# Autodesk Inventor assembly: TS_V1_Fallmagazin_gesamt
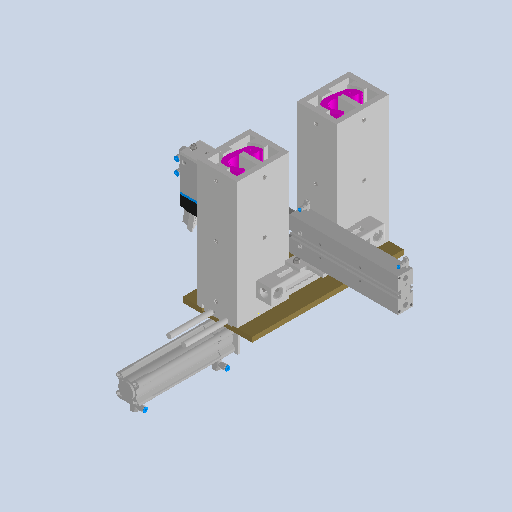
[picture p0: Inventor's stored thumbnail of the model, 512x512]
Saved by Autodesk Inventor 2025.2 (Build 292293000, 293)
## iProperties
Created: 2025-06-10
Part Number: TS_V1_Fallmagazin_gesamt
Document SubType Name: Assembly
Designer: tino
Author: tino
## Documents named in this file (36)
- D:\Useless_Box\CAD-Paspa\Useless Box\Eigene Bauteile\Fallmagazin\TS_V1_Fallmagazin_gesamt.iam
- D:\Useless_Box\CAD-Paspa\Useless Box\Eigene Bauteile\Fallmagazin\TS_V1_Fallmagazin_Boden_int.ipt
- D:\Useless_Box\CAD-Paspa\Useless Box\Eigene Bauteile\Fallmagazin\TS_V1_Fallmagazin_Wandung_int.ipt
- D:\Useless_Box\CAD-Paspa\Useless Box\Eigene Bauteile\Fallmagazin\TS_V1_Fallmagazin_Leitbleche_vorne_int.ipt
- D:\Useless_Box\CAD-Paspa\Useless Box\_Useless_Box\Finger.ipt
- D:\Useless_Box\CAD-Paspa\Useless Box\Eigene Bauteile\Fallmagazin\TS_V1_Fallmagazin_Schieber.iam
- D:\Useless_Box\CAD-Paspa\Useless Box\Kaufteile\Festo_Normzylinder_100\1376426 DSBC-32-100-PPVA-N3---(0).iam
- D:\Useless_Box\CAD-Paspa\Useless Box\Standart Bauteile\ISO 4762 - M4 x 12ISO.ipt
- D:\Useless_Box\CAD-Paspa\Useless Box\Standart Bauteile\ISO 4762 - M4 x 16ISO.ipt
- D:\Useless_Box\CAD-Paspa\Useless Box\Eigene Bauteile\Fallmagazin\TS_V1_Fallmagazin_Zylinderanbindung_int.ipt
- D:\Useless_Box\CAD-Paspa\Useless Box\Eigene Bauteile\Fallmagazin\TS_V1_Fallmagazin_Stopper_int.ipt
- D:\Useless_Box\CAD-Paspa\Useless Box\Eigene Bauteile\Fallmagazin\TS_V1_Fallmagazin_Zylinderhalter_int.ipt
- D:\Useless_Box\CAD-Paspa\Useless Box\Standart Bauteile\ISO 4762 - M5 x 8ISO.ipt
- D:\Useless_Box\CAD-Paspa\Useless Box\Standart Bauteile\ISO 4762 - M5 x 20ISO.ipt
- D:\Useless_Box\CAD-Paspa\Useless Box\Standart Bauteile\DIN EN ISO 2338 - 4 m6 x 10.ipt
- D:\Useless_Box\CAD-Paspa\Useless Box\Standart Bauteile\DIN 7991 - M5x12.ipt
- D:\Useless_Box\CAD-Paspa\Useless Box\Eigene Bauteile\Fallmagazin\TS_V1_Fallmagazin_Schieberanbindung_int.ipt
- D:\Useless_Box\CAD-Paspa\Useless Box\Eigene Bauteile\Fallmagazin\TS_V1_Fallmagazin_Verbindungsstange_int.ipt
- D:\Useless_Box\CAD-Paspa\Useless Box\Kaufteile\Festo_Fuehrungszylinder150_DFM_16\529120 DFM-16-150-B-P-A-KF---(0).iam
- D:\Useless_Box\CAD-Paspa\Useless Box\Kaufteile\DHRS-32-A - Kopie\AIS2024\1310164 DHRS-32-A---(0).iam
- D:\Useless_Box\CAD-Paspa\Useless Box\Eigene Bauteile\TS_Adapter_Greifer_int.ipt
- D:\Useless_Box\CAD-Paspa\Useless Box\Standart Bauteile\ISO 4762 - M4 x 10ISO.ipt
- D:\Useless_Box\CAD-Paspa\Useless Box\Eigene Bauteile\TS_Halterung_Fuehrungszylinder_int.ipt
- D:\Useless_Box\CAD-Paspa\Useless Box\Kaufteile\Rexroth_Profil+Winkel_30x30\Rexroth_30x30_Wuerfel\Rexroth_30x30_Wuerfel\Rexroth_30x30_Wuerfel.ipt
- D:\Useless_Box\CAD-Paspa\Useless Box\Kaufteile\Rexroth_Profil+Winkel_30x30\Rexroth_30x30_200_ext\Rexroth_30x30_200_ext\Rexroth_30x30_200_ext.ipt
- D:\Useless_Box\CAD-Paspa\Useless Box\Standart Bauteile\DIN 7991 - M8x16.ipt
- D:\Useless_Box\CAD-Paspa\Useless Box\Standart Bauteile\DIN 934 - M5 x 0,8.ipt
- D:\Useless_Box\CAD-Paspa\Useless Box\Standart Bauteile\ISO 4762 - M6 x 12ISO.ipt
- D:\Useless_Box\CAD-Paspa\Useless Box\Kaufteile\Rexroth_Hammermuttern\Rexroth_Hammermutter_8_M6\Rexroth_Hammermutter_8_M6\Rexroth_Hammermutter_8_M6.ipt
- D:\Useless_Box\CAD-Paspa\Useless Box\Standart Bauteile\DIN 913 - M5 x 6.ipt
- D:\Useless_Box\CAD-Paspa\Useless Box\Eigene Bauteile\JH_Greifer_Unterlegscheibe\Kaufteile\Drosselrückschlagventil\175043 GRLZ-M3-QS-3.ipt
- D:\Useless_Box\CAD-Paspa\Useless Box\Eigene Bauteile\JH_Greifer_Unterlegscheibe\Kaufteile\Drosselrückschlagventil\193143 GRLA-1_8-QS-4-D.ipt
- D:\Useless_Box\CAD-Paspa\Useless Box\Standart Bauteile\DIN 6912 - M4 x 10.ipt
- C:\Users\Erik\Documents\Inventor\Content Center Files\R2025\de-DE\DIN ISO 8734(1)\ISO 8734 - 4 x 10 - ADIN EN.ipt
- D:\Useless_Box\CAD-Paspa\Useless Box\Standart Bauteile\DIN EN ISO 4762 - M5 x 10.ipt
- D:\Useless_Box\CAD-Paspa\Useless Box\Standart Bauteile\DIN 125 - A 5,3.ipt
## Components (206 placed, 35 different names)
1. TS_V1_Fallmagazin_Boden_int:1 — Passend:16, Passend:17, Passend:21, Passend:23, Passend:25, Passend:26, Passend:30, Passend:43, Passend:44, Passend:45, Passend:46, Fluchtend:18, Passend:84, Passend:85, Passend:86, Passend:87, Passend:94, Passend:96, Passend:97, Fluchtend:19, Fluchtend:20, Passend:121, Winkel:11, Winkel:12
2. TS_V1_Fallmagazin_Wandung_int:2 — Passend:7, Passend:8, Fluchtend:4, Winkel:1, Winkel:2, Passend:16, Passend:17, Passend:35, Passend:36, Passend:37, Passend:38, Passend:39, Passend:40, Passend:41, Passend:42, Winkel:3, Passend:130
3. TS_V1_Fallmagazin_Leitbleche_vorne_int:1 — Passend:7, Passend:8, Fluchtend:4, Tangential:2, Tangential:5, Fluchtend:12
4. TS_V1_Fallmagazin_Schieber:1 [sub-assembly] — Passend:21, Passend:25, Passend:26, Passend:53, Passend:61, Passend:62, Passend:63, Passend:64, Passend:106, Tangential:6
5. TS_V1_Fallmagazin_Schieber:2 [sub-assembly] — Passend:23, Passend:30, Passend:65, Passend:66, Passend:67, Passend:101, Passend:103, Passend:107
6. 1376426 DSBC-32-100-PPVA-N3---(0):1 [sub-assembly] — Fluchtend:18, Passend:68, Passend:69, Passend:92, Passend:93, Passend:99, Einfügen:1, Passend:159
7. TS_V1_Fallmagazin_Wandung_int:3 — Passend:45, Passend:46, Passend:47, Fluchtend:14, Passend:48, Passend:132, Passend:137, Passend:138
8. TS_V1_Fallmagazin_Leitbleche_vorne_int:2 — Passend:47, Fluchtend:14, Passend:48
9. TS_V1_Fallmagazin_Zylinderanbindung_int:1 — Passend:53, Passend:99, Winkel:4, Passend:104, Passend:108, Passend:110, Passend:144
10. TS_V1_Fallmagazin_Stopper_int:1 — Passend:61, Passend:62, Winkel:3
11. TS_V1_Fallmagazin_Stopper_int:2 — Passend:63, Passend:64
12. TS_V1_Fallmagazin_Stopper_int:3 — Passend:65, Fluchtend:16, Passend:67
13. TS_V1_Fallmagazin_Stopper_int:4 — Passend:66, Fluchtend:16
14. TS_V1_Fallmagazin_Zylinderhalter_int:1 — Passend:68, Passend:69, Passend:71, Passend:72, Passend:90, Passend:91, Passend:93, Passend:95, Passend:97
15. DIN 7991 M5x12:1 — Passend:106, Tangential:6, Passend:108
16. DIN 7991 M5x12:2 — Passend:101, Passend:107, Passend:109
17. TS_V1_Fallmagazin_Schieberanbindung_int:1 — Winkel:4, Passend:103, Passend:105, Passend:109, Passend:142
18. TS_V1_Fallmagazin_Verbindungsstange_int:1 — Passend:104, Passend:105, Winkel:5, Passend:110, Passend:141, Passend:143
19. 529120 DFM-16-150-B-P-A-KF---(0):1 [sub-assembly] — Fluchtend:19, Winkel:6, Fluchtend:21, Passend:116, Passend:117, Passend:120, Passend:121, Passend:122, Passend:123, Passend:124, Winkel:7, Winkel:8, Passend:157, Passend:158, Winkel:10
20. 1310164 DHRS-32-A---(0):1 [sub-assembly] — Fluchtend:20, Fluchtend:21, Passend:113, Passend:118, Passend:119, Passend:153, Passend:155, Passend:156, Einfügen:2, Einfügen:3, Einfügen:4, Einfügen:5, Einfügen:6, Einfügen:7, Passend:162
21. TS_Adapter_Greifer_int:1 — Passend:113, Passend:114, Passend:115, Passend:118, Passend:119, Passend:120, Passend:153, Passend:154, Fluchtend:26, Winkel:9, Passend:163
22. TS_Halterung_Fuehrungszylinder_int:1 — Passend:122, Passend:123, Passend:124, Passend:135, Passend:145, Passend:146, Passend:147, Passend:148, Passend:150, Passend:151, Passend:152
23. Rexroth_30x30_Wuerfel:1 — Passend:130, Passend:134, Fluchtend:24, Fluchtend:25, Passend:136, Tangential:7, Passend:139, Tangential:9
24. Rexroth_30x30_Wuerfel:2 — Passend:132, Passend:133, Fluchtend:22, Fluchtend:23, Passend:137, Tangential:8, Passend:140, Tangential:10
25. Rexroth_30x30_170_ext:1 — Passend:133, Fluchtend:22, Fluchtend:23, Passend:134, Fluchtend:24, Fluchtend:25, Passend:135, Tangential:11, Tangential:12
26. DIN 7991 M8x16:3 — Passend:136, Tangential:7
27. DIN 7991 M8x16:4 — Passend:138, Tangential:8
28. DIN 7991 M8x16:5 — Passend:139, Tangential:9
29. DIN 7991 M8x16:6 — Passend:140, Tangential:10
30. DIN 934 - M5 x 0,8:1 — Passend:141, Passend:142
31. DIN 934 - M5 x 0,8:2 — Passend:143, Passend:144
32. ISO 4762 - M6 x 12ISO:1 — Passend:147, Passend:148, Passend:149
33. Rexroth_Hammermutter_8_M6:1 — Winkel:7, Tangential:11, Passend:149
34. Rexroth_Hammermutter_8_M6:2 — Winkel:8, Tangential:12, Passend:150
35. ISO 4762 - M6 x 12ISO:2 — Passend:151, Passend:152
36. DIN 913 - M5 x 6:1 — Passend:154, Fluchtend:26
37. 193143 GRLA-1_8-QS-4-D:3 — Einfügen:1, Winkel:11
38. 193143 GRLA-1_8-QS-4-D:4 — Passend:159, Winkel:12
39. DIN 6912 - M4 x 10:1 — Einfügen:2
40. DIN 6912 - M4 x 10:2 — Einfügen:3
41. DIN 6912 - M4 x 10:3 — Einfügen:4
42. DIN 6912 - M4 x 10:4 — Einfügen:5
43. DIN EN ISO 8734 4 x 10 - A:1 — Einfügen:7
44. DIN EN ISO 8734 4 x 10 - A:2 — Einfügen:6
45. Finger:1 — Winkel:1, Tangential:2, Tangential:5, Winkel:2, Fluchtend:12
46. Finger:2
47. Finger:3
48. Finger:4
49. Finger:5
50. Finger:6
51. Finger:7
52. Finger:8
53. Finger:9
54. Finger:10
55. Finger:11
56. Finger:12
57. Finger:13
58. Finger:14
59. Finger:15
60. Finger:16
61. Finger:17
62. Finger:18
63. Finger:19
64. Finger:20
65. Finger:21
66. Finger:22
67. Finger:23
68. Finger:24
69. Finger:25
70. Finger:26
71. Finger:27
72. Finger:28
73. Finger:29
74. Finger:30
75. Finger:31
76. Finger:32
77. Finger:33
78. Finger:34
79. Finger:35
80. Finger:36
81. Finger:37
82. Finger:38
83. Finger:39
84. Finger:40
85. Finger:41
86. Finger:42
87. Finger:43
88. Finger:44
89. Finger:45
90. Finger:46
91. Finger:47
92. Finger:48
93. Finger:49
94. Finger:50
95. Finger:51
96. Finger:52
97. Finger:53
98. Finger:54
99. Finger:55
100. Finger:56
101. Finger:57
102. Finger:58
103. Finger:59
104. Finger:60
105. Finger:61
106. Finger:62
107. Finger:63
108. Finger:64
109. Finger:65
110. Finger:66
111. Finger:67
112. Finger:68
113. Finger:69
114. Finger:70
115. Finger:71
116. Finger:72
117. Finger:73
118. Finger:74
119. Finger:75
120. Finger:76
121. Finger:77
122. Finger:78
123. Finger:79
124. Finger:80
125. Finger:81
126. Finger:82
127. Finger:83
128. Finger:84
129. Finger:85
130. Finger:86
131. Finger:87
132. Finger:88
133. Finger:89
134. Finger:90
135. Finger:91
136. Finger:92
137. Finger:93
138. Finger:94
139. Finger:95
140. Finger:96
141. Finger:97
142. Finger:98
143. ISO 4762 M5 x 8:1 — Passend:71, Passend:72, Passend:96
144. ISO 4762 M5 x 8:2
145. ISO 4762 M5 x 8:3 — Passend:94
146. ISO 4762 M5 x 8:4
147. ISO 4762 M5 x 20:1 — Passend:92, Passend:95
148. ISO 4762 M5 x 20:2 — Passend:91
149. ISO 4762 M5 x 20:3 — Passend:90
150. ISO 4762 M5 x 20:4
151. ISO 4762 M4 x 10:1 — Passend:114, Passend:115, Passend:116
152. ISO 4762 M4 x 10:2 — Passend:117
153. ISO 4762 M4 x 10:3
154. ISO 4762 M4 x 10:4
155. DIN EN ISO 2338 4 m6 x 10:1 — Passend:84, Passend:85
156. DIN EN ISO 2338 4 m6 x 10:2 — Passend:86, Passend:87
157. DIN EN ISO 2338 4 m6 x 10:3
158. DIN EN ISO 2338 4 m6 x 10:4
159. ISO 4762 M4 x 10:5 — Passend:145, Passend:146
160. ISO 4762 M4 x 10:6
161. ISO 4762 M4 x 10:7
162. ISO 4762 M4 x 10:8
163. 193143 GRLA-1_8-QS-4-D:1 — Passend:155, Passend:156, Winkel:9
164. 193143 GRLA-1_8-QS-4-D:2
165. 175043 GRLZ-M3-QS-3:1 — Passend:157, Passend:158, Winkel:10
166. 175043 GRLZ-M3-QS-3:2
167. DIN 125 - A 5,3:1 — Passend:163
168. DIN EN ISO 4762 - M5 x 10:1 — Passend:162
169. DIN 125 - A 5,3:2
170. DIN EN ISO 4762 - M5 x 10:2
171. ISO 4762 M4 x 12:1 — Passend:35, Passend:36
172. ISO 4762 M4 x 12:2
173. ISO 4762 M4 x 12:3
174. ISO 4762 M4 x 12:4 — Passend:37, Passend:38
175. ISO 4762 M4 x 12:5
176. ISO 4762 M4 x 12:6
177. ISO 4762 M4 x 12:7 — Passend:39, Passend:40
178. ISO 4762 M4 x 12:8
179. ISO 4762 M4 x 12:9
180. ISO 4762 M4 x 12:10 — Passend:41, Passend:42
181. ISO 4762 M4 x 12:11
182. ISO 4762 M4 x 12:12
183. ISO 4762 M4 x 16:1 — Passend:43, Passend:44
184. ISO 4762 M4 x 16:2
185. ISO 4762 M4 x 16:3
186. ISO 4762 M4 x 16:4
187. ISO 4762 M4 x 16:5
188. ISO 4762 M4 x 16:6
189. ISO 4762 M4 x 12:13
190. ISO 4762 M4 x 12:14
191. ISO 4762 M4 x 12:15
192. ISO 4762 M4 x 12:16
193. ISO 4762 M4 x 12:17
194. ISO 4762 M4 x 12:18
195. ISO 4762 M4 x 12:19
196. ISO 4762 M4 x 12:20
197. ISO 4762 M4 x 12:21
198. ISO 4762 M4 x 12:22
199. ISO 4762 M4 x 12:23
200. ISO 4762 M4 x 12:24
201. ISO 4762 M4 x 16:7
202. ISO 4762 M4 x 16:8
203. ISO 4762 M4 x 16:9
204. ISO 4762 M4 x 16:10
205. ISO 4762 M4 x 16:11
206. ISO 4762 M4 x 16:12
## Component patterns: (2 elements), (98 elements, first: Finger:1), (4 elements, first: ISO 4762 M5 x 8:1), (4 elements, first: ISO 4762 M5 x 20:1), (4 elements, first: ISO 4762 M4 x 10:1), (2 elements, first: DIN EN ISO 2338 4 m6 x 10:1 + DIN EN ISO 2338 4 m6 x 10:2), (4 elements, first: ISO 4762 M4 x 10:5), (2 elements, first: 193143 GRLA-1_8-QS-4-D:1), (2 elements, first: 175043 GRLZ-M3-QS-3:1), (2 elements, first: DIN 125 - A 5,3:1 + DIN EN ISO 4762 - M5 x 10:1), (3 elements, first: ISO 4762 M4 x 12:1), (3 elements, first: ISO 4762 M4 x 12:4), (3 elements, first: ISO 4762 M4 x 12:7), (3 elements, first: ISO 4762 M4 x 12:10), (6 elements, first: ISO 4762 M4 x 16:1), Komponentenanordnung 2:2 (3 elements), Komponentenanordnung 3:2 (3 elements), Komponentenanordnung 4:2 (3 elements), Komponentenanordnung 5:2 (3 elements), Komponentenanordnung 6:2 (6 elements)
## Relationships (143: Mate 102, Flush 13, Angle 12, Tangent 9, Insert 7)
- Passend:7 [Mate]: TS_V1_Fallmagazin_Wandung_int:2 ↔ TS_V1_Fallmagazin_Leitbleche_vorne_int:1
- Passend:8 [Mate]: TS_V1_Fallmagazin_Wandung_int:2 ↔ TS_V1_Fallmagazin_Leitbleche_vorne_int:1
- Fluchtend:4 [Flush]: TS_V1_Fallmagazin_Wandung_int:2 ↔ TS_V1_Fallmagazin_Leitbleche_vorne_int:1
- Winkel:1 [Angle] (0 deg): TS_V1_Fallmagazin_Wandung_int:2 ↔ Finger:1
- Tangential:2: TS_V1_Fallmagazin_Leitbleche_vorne_int:1 ↔ Finger:1
- Tangential:5: TS_V1_Fallmagazin_Leitbleche_vorne_int:1 ↔ Finger:1
- Winkel:2 [Angle] (0 deg): TS_V1_Fallmagazin_Wandung_int:2 ↔ Finger:1
- Passend:16 [Mate]: TS_V1_Fallmagazin_Boden_int:1 ↔ TS_V1_Fallmagazin_Wandung_int:2
- Passend:17 [Mate]: TS_V1_Fallmagazin_Boden_int:1 ↔ TS_V1_Fallmagazin_Wandung_int:2
- Passend:21 [Mate]: TS_V1_Fallmagazin_Boden_int:1 ↔ TS_V1_Fallmagazin_Schieber:1
- Passend:23 [Mate]: TS_V1_Fallmagazin_Boden_int:1 ↔ TS_V1_Fallmagazin_Schieber:2
- Passend:25 [Mate]: TS_V1_Fallmagazin_Boden_int:1 ↔ TS_V1_Fallmagazin_Schieber:1
- Passend:26 [Mate]: TS_V1_Fallmagazin_Boden_int:1 ↔ TS_V1_Fallmagazin_Schieber:1
- Passend:30 [Mate]: TS_V1_Fallmagazin_Boden_int:1 ↔ TS_V1_Fallmagazin_Schieber:2
- Passend:35 [Mate]: TS_V1_Fallmagazin_Wandung_int:2 ↔ ISO 4762 M4 x 12:1
- Passend:36 [Mate]: TS_V1_Fallmagazin_Wandung_int:2 ↔ ISO 4762 M4 x 12:1
- Passend:37 [Mate]: TS_V1_Fallmagazin_Wandung_int:2 ↔ ISO 4762 M4 x 12:4
- Passend:38 [Mate]: TS_V1_Fallmagazin_Wandung_int:2 ↔ ISO 4762 M4 x 12:4
- Passend:39 [Mate]: TS_V1_Fallmagazin_Wandung_int:2 ↔ ISO 4762 M4 x 12:7
- Passend:40 [Mate]: TS_V1_Fallmagazin_Wandung_int:2 ↔ ISO 4762 M4 x 12:7
- Passend:41 [Mate]: TS_V1_Fallmagazin_Wandung_int:2 ↔ ISO 4762 M4 x 12:10
- Passend:42 [Mate]: TS_V1_Fallmagazin_Wandung_int:2 ↔ ISO 4762 M4 x 12:10
- Passend:43 [Mate]: TS_V1_Fallmagazin_Boden_int:1 ↔ ISO 4762 M4 x 16:1
- Passend:44 [Mate]: TS_V1_Fallmagazin_Boden_int:1 ↔ ISO 4762 M4 x 16:1
- Fluchtend:12 [Flush]: TS_V1_Fallmagazin_Leitbleche_vorne_int:1 ↔ Finger:1
- Passend:45 [Mate]: TS_V1_Fallmagazin_Boden_int:1 ↔ TS_V1_Fallmagazin_Wandung_int:3
- Passend:46 [Mate]: TS_V1_Fallmagazin_Boden_int:1 ↔ TS_V1_Fallmagazin_Wandung_int:3
- Passend:47 [Mate]: TS_V1_Fallmagazin_Wandung_int:3 ↔ TS_V1_Fallmagazin_Leitbleche_vorne_int:2
- Fluchtend:14 [Flush]: TS_V1_Fallmagazin_Wandung_int:3 ↔ TS_V1_Fallmagazin_Leitbleche_vorne_int:2
- Passend:48 [Mate]: TS_V1_Fallmagazin_Wandung_int:3 ↔ TS_V1_Fallmagazin_Leitbleche_vorne_int:2
- Passend:53 [Mate]: TS_V1_Fallmagazin_Schieber:1 ↔ TS_V1_Fallmagazin_Zylinderanbindung_int:1
- Passend:61 [Mate]: TS_V1_Fallmagazin_Schieber:1 ↔ TS_V1_Fallmagazin_Stopper_int:1
- Passend:62 [Mate]: TS_V1_Fallmagazin_Schieber:1 ↔ TS_V1_Fallmagazin_Stopper_int:1
- Passend:63 [Mate]: TS_V1_Fallmagazin_Schieber:1 ↔ TS_V1_Fallmagazin_Stopper_int:2
- Passend:64 [Mate]: TS_V1_Fallmagazin_Schieber:1 ↔ TS_V1_Fallmagazin_Stopper_int:2
- Passend:65 [Mate]: TS_V1_Fallmagazin_Schieber:2 ↔ TS_V1_Fallmagazin_Stopper_int:3
- Passend:66 [Mate]: TS_V1_Fallmagazin_Schieber:2 ↔ TS_V1_Fallmagazin_Stopper_int:4
- Fluchtend:16 [Flush]: TS_V1_Fallmagazin_Stopper_int:3 ↔ TS_V1_Fallmagazin_Stopper_int:4
- Passend:67 [Mate]: TS_V1_Fallmagazin_Schieber:2 ↔ TS_V1_Fallmagazin_Stopper_int:3
- Fluchtend:18 [Flush]: TS_V1_Fallmagazin_Boden_int:1 ↔ 1376426 DSBC-32-100-PPVA-N3---(0):1
- Passend:68 [Mate]: 1376426 DSBC-32-100-PPVA-N3---(0):1 ↔ TS_V1_Fallmagazin_Zylinderhalter_int:1
- Passend:69 [Mate]: 1376426 DSBC-32-100-PPVA-N3---(0):1 ↔ TS_V1_Fallmagazin_Zylinderhalter_int:1
- Passend:71 [Mate]: TS_V1_Fallmagazin_Zylinderhalter_int:1 ↔ ISO 4762 M5 x 8:1
- Passend:72 [Mate]: TS_V1_Fallmagazin_Zylinderhalter_int:1 ↔ ISO 4762 M5 x 8:1
- Passend:84 [Mate]: TS_V1_Fallmagazin_Boden_int:1 ↔ DIN EN ISO 2338 4 m6 x 10:1
- Passend:85 [Mate] (0.5 mm): TS_V1_Fallmagazin_Boden_int:1 ↔ DIN EN ISO 2338 4 m6 x 10:1
- Passend:86 [Mate]: TS_V1_Fallmagazin_Boden_int:1 ↔ DIN EN ISO 2338 4 m6 x 10:2
- Passend:87 [Mate] (1 mm): TS_V1_Fallmagazin_Boden_int:1 ↔ DIN EN ISO 2338 4 m6 x 10:2
- Winkel:3 [Angle] (0 deg): TS_V1_Fallmagazin_Wandung_int:2 ↔ TS_V1_Fallmagazin_Stopper_int:1
- Passend:90 [Mate]: TS_V1_Fallmagazin_Zylinderhalter_int:1 ↔ ISO 4762 M5 x 20:3
- Passend:91 [Mate]: TS_V1_Fallmagazin_Zylinderhalter_int:1 ↔ ISO 4762 M5 x 20:2
- Passend:92 [Mate]: 1376426 DSBC-32-100-PPVA-N3---(0):1 ↔ ISO 4762 M5 x 20:1
- Passend:93 [Mate]: 1376426 DSBC-32-100-PPVA-N3---(0):1 ↔ TS_V1_Fallmagazin_Zylinderhalter_int:1
- Passend:94 [Mate]: TS_V1_Fallmagazin_Boden_int:1 ↔ ISO 4762 M5 x 8:3
- Passend:95 [Mate]: TS_V1_Fallmagazin_Zylinderhalter_int:1 ↔ ISO 4762 M5 x 20:1
- Passend:96 [Mate]: TS_V1_Fallmagazin_Boden_int:1 ↔ ISO 4762 M5 x 8:1
- Passend:97 [Mate]: TS_V1_Fallmagazin_Boden_int:1 ↔ TS_V1_Fallmagazin_Zylinderhalter_int:1
- Passend:99 [Mate]: 1376426 DSBC-32-100-PPVA-N3---(0):1 ↔ TS_V1_Fallmagazin_Zylinderanbindung_int:1
- Passend:101 [Mate]: TS_V1_Fallmagazin_Schieber:2 ↔ DIN 7991 M5x12:2
- Winkel:4 [Angle] (180 deg): TS_V1_Fallmagazin_Zylinderanbindung_int:1 ↔ TS_V1_Fallmagazin_Schieberanbindung_int:1
- Passend:103 [Mate]: TS_V1_Fallmagazin_Schieber:2 ↔ TS_V1_Fallmagazin_Schieberanbindung_int:1
- Passend:104 [Mate]: TS_V1_Fallmagazin_Zylinderanbindung_int:1 ↔ TS_V1_Fallmagazin_Verbindungsstange_int:1
- Passend:105 [Mate] (-10 mm): TS_V1_Fallmagazin_Schieberanbindung_int:1 ↔ TS_V1_Fallmagazin_Verbindungsstange_int:1
- Winkel:5 [Angle] (0 deg): TS_V1_Fallmagazin_Verbindungsstange_int:1
- Passend:106 [Mate]: TS_V1_Fallmagazin_Schieber:1 ↔ DIN 7991 M5x12:1
- Tangential:6: TS_V1_Fallmagazin_Schieber:1 ↔ DIN 7991 M5x12:1
- Passend:107 [Mate]: TS_V1_Fallmagazin_Schieber:2 ↔ DIN 7991 M5x12:2
- Passend:108 [Mate]: TS_V1_Fallmagazin_Zylinderanbindung_int:1 ↔ DIN 7991 M5x12:1
- Passend:109 [Mate]: DIN 7991 M5x12:2 ↔ TS_V1_Fallmagazin_Schieberanbindung_int:1
- Passend:110 [Mate] (-10 mm): TS_V1_Fallmagazin_Zylinderanbindung_int:1 ↔ TS_V1_Fallmagazin_Verbindungsstange_int:1
- Fluchtend:19 [Flush] (22.694 mm): TS_V1_Fallmagazin_Boden_int:1 ↔ 529120 DFM-16-150-B-P-A-KF---(0):1
- Winkel:6 [Angle] (0 deg): 529120 DFM-16-150-B-P-A-KF---(0):1
- Fluchtend:20 [Flush] (-135 mm): TS_V1_Fallmagazin_Boden_int:1 ↔ 1310164 DHRS-32-A---(0):1
- Fluchtend:21 [Flush]: 529120 DFM-16-150-B-P-A-KF---(0):1 ↔ 1310164 DHRS-32-A---(0):1
- Passend:113 [Mate]: 1310164 DHRS-32-A---(0):1 ↔ TS_Adapter_Greifer_int:1
- Passend:114 [Mate]: TS_Adapter_Greifer_int:1 ↔ ISO 4762 M4 x 10:1
- Passend:115 [Mate]: TS_Adapter_Greifer_int:1 ↔ ISO 4762 M4 x 10:1
- Passend:116 [Mate]: 529120 DFM-16-150-B-P-A-KF---(0):1 ↔ ISO 4762 M4 x 10:1
- Passend:117 [Mate]: 529120 DFM-16-150-B-P-A-KF---(0):1 ↔ ISO 4762 M4 x 10:2
- Passend:118 [Mate]: 1310164 DHRS-32-A---(0):1 ↔ TS_Adapter_Greifer_int:1
- Passend:119 [Mate]: 1310164 DHRS-32-A---(0):1 ↔ TS_Adapter_Greifer_int:1
- Passend:120 [Mate]: 529120 DFM-16-150-B-P-A-KF---(0):1 ↔ TS_Adapter_Greifer_int:1
- Passend:121 [Mate] (30.575 mm): TS_V1_Fallmagazin_Boden_int:1 ↔ 529120 DFM-16-150-B-P-A-KF---(0):1
- Passend:122 [Mate]: 529120 DFM-16-150-B-P-A-KF---(0):1 ↔ TS_Halterung_Fuehrungszylinder_int:1
- Passend:123 [Mate]: 529120 DFM-16-150-B-P-A-KF---(0):1 ↔ TS_Halterung_Fuehrungszylinder_int:1
- Passend:124 [Mate]: 529120 DFM-16-150-B-P-A-KF---(0):1 ↔ TS_Halterung_Fuehrungszylinder_int:1
- Passend:130 [Mate]: TS_V1_Fallmagazin_Wandung_int:2 ↔ Rexroth_30x30_Wuerfel:1
- Passend:132 [Mate]: TS_V1_Fallmagazin_Wandung_int:3 ↔ Rexroth_30x30_Wuerfel:2
- Passend:133 [Mate]: Rexroth_30x30_Wuerfel:2 ↔ Rexroth_30x30_170_ext:1
- Fluchtend:22 [Flush]: Rexroth_30x30_Wuerfel:2 ↔ Rexroth_30x30_170_ext:1
- Fluchtend:23 [Flush]: Rexroth_30x30_Wuerfel:2 ↔ Rexroth_30x30_170_ext:1
- Passend:134 [Mate]: Rexroth_30x30_Wuerfel:1 ↔ Rexroth_30x30_170_ext:1
- Fluchtend:24 [Flush]: Rexroth_30x30_Wuerfel:1 ↔ Rexroth_30x30_170_ext:1
- Fluchtend:25 [Flush]: Rexroth_30x30_Wuerfel:1 ↔ Rexroth_30x30_170_ext:1
- Passend:135 [Mate]: TS_Halterung_Fuehrungszylinder_int:1 ↔ Rexroth_30x30_170_ext:1
- Passend:136 [Mate]: Rexroth_30x30_Wuerfel:1 ↔ DIN 7991 M8x16:3
- Tangential:7: Rexroth_30x30_Wuerfel:1 ↔ DIN 7991 M8x16:3
- Passend:137 [Mate]: TS_V1_Fallmagazin_Wandung_int:3 ↔ Rexroth_30x30_Wuerfel:2
- Passend:138 [Mate]: TS_V1_Fallmagazin_Wandung_int:3 ↔ DIN 7991 M8x16:4
- Tangential:8: Rexroth_30x30_Wuerfel:2 ↔ DIN 7991 M8x16:4
- Passend:139 [Mate]: Rexroth_30x30_Wuerfel:1 ↔ DIN 7991 M8x16:5
- Tangential:9: Rexroth_30x30_Wuerfel:1 ↔ DIN 7991 M8x16:5
- Passend:140 [Mate]: Rexroth_30x30_Wuerfel:2 ↔ DIN 7991 M8x16:6
- Tangential:10: Rexroth_30x30_Wuerfel:2 ↔ DIN 7991 M8x16:6
- Passend:141 [Mate]: TS_V1_Fallmagazin_Verbindungsstange_int:1 ↔ DIN 934 - M5 x 0,8:1
- Passend:142 [Mate]: TS_V1_Fallmagazin_Schieberanbindung_int:1 ↔ DIN 934 - M5 x 0,8:1
- Passend:143 [Mate]: TS_V1_Fallmagazin_Verbindungsstange_int:1 ↔ DIN 934 - M5 x 0,8:2
- Passend:144 [Mate]: TS_V1_Fallmagazin_Zylinderanbindung_int:1 ↔ DIN 934 - M5 x 0,8:2
- Passend:145 [Mate]: TS_Halterung_Fuehrungszylinder_int:1 ↔ ISO 4762 M4 x 10:5
- Passend:146 [Mate]: TS_Halterung_Fuehrungszylinder_int:1 ↔ ISO 4762 M4 x 10:5
- Passend:147 [Mate]: TS_Halterung_Fuehrungszylinder_int:1 ↔ ISO 4762 - M6 x 12ISO:1
- Passend:148 [Mate]: TS_Halterung_Fuehrungszylinder_int:1 ↔ ISO 4762 - M6 x 12ISO:1
- Winkel:7 [Angle] (180 deg): 529120 DFM-16-150-B-P-A-KF---(0):1 ↔ Rexroth_Hammermutter_8_M6:1
- Tangential:11: Rexroth_30x30_170_ext:1 ↔ Rexroth_Hammermutter_8_M6:1
- Passend:149 [Mate]: ISO 4762 - M6 x 12ISO:1 ↔ Rexroth_Hammermutter_8_M6:1
- Winkel:8 [Angle] (0 deg): 529120 DFM-16-150-B-P-A-KF---(0):1 ↔ Rexroth_Hammermutter_8_M6:2
- Tangential:12: Rexroth_30x30_170_ext:1 ↔ Rexroth_Hammermutter_8_M6:2
- Passend:150 [Mate]: TS_Halterung_Fuehrungszylinder_int:1 ↔ Rexroth_Hammermutter_8_M6:2
- Passend:151 [Mate]: TS_Halterung_Fuehrungszylinder_int:1 ↔ ISO 4762 - M6 x 12ISO:2
- Passend:152 [Mate]: TS_Halterung_Fuehrungszylinder_int:1 ↔ ISO 4762 - M6 x 12ISO:2
- Passend:153 [Mate]: 1310164 DHRS-32-A---(0):1 ↔ TS_Adapter_Greifer_int:1
- Passend:154 [Mate]: TS_Adapter_Greifer_int:1 ↔ DIN 913 - M5 x 6:1
- Fluchtend:26 [Flush]: TS_Adapter_Greifer_int:1 ↔ DIN 913 - M5 x 6:1
- Passend:155 [Mate]: 1310164 DHRS-32-A---(0):1 ↔ 193143 GRLA-1_8-QS-4-D:1
- Passend:156 [Mate]: 1310164 DHRS-32-A---(0):1 ↔ 193143 GRLA-1_8-QS-4-D:1
- Winkel:9 [Angle] (0 deg): TS_Adapter_Greifer_int:1 ↔ 193143 GRLA-1_8-QS-4-D:1
- Passend:157 [Mate]: 529120 DFM-16-150-B-P-A-KF---(0):1 ↔ 175043 GRLZ-M3-QS-3:1
- Passend:158 [Mate]: 529120 DFM-16-150-B-P-A-KF---(0):1 ↔ 175043 GRLZ-M3-QS-3:1
- Winkel:10 [Angle] (180 deg): 529120 DFM-16-150-B-P-A-KF---(0):1 ↔ 175043 GRLZ-M3-QS-3:1
- Einfügen:1 [Insert]: 1376426 DSBC-32-100-PPVA-N3---(0):1 ↔ 193143 GRLA-1_8-QS-4-D:3
- Winkel:11 [Angle] (0 deg): TS_V1_Fallmagazin_Boden_int:1 ↔ 193143 GRLA-1_8-QS-4-D:3
- Passend:159 [Mate]: 1376426 DSBC-32-100-PPVA-N3---(0):1 ↔ 193143 GRLA-1_8-QS-4-D:4
- Winkel:12 [Angle] (0 deg): TS_V1_Fallmagazin_Boden_int:1 ↔ 193143 GRLA-1_8-QS-4-D:4
- Einfügen:2 [Insert]: 1310164 DHRS-32-A---(0):1 ↔ DIN 6912 - M4 x 10:1
- Einfügen:3 [Insert]: 1310164 DHRS-32-A---(0):1 ↔ DIN 6912 - M4 x 10:2
- Einfügen:4 [Insert]: 1310164 DHRS-32-A---(0):1 ↔ DIN 6912 - M4 x 10:3
- Einfügen:5 [Insert]: 1310164 DHRS-32-A---(0):1 ↔ DIN 6912 - M4 x 10:4
- Einfügen:6 [Insert]: 1310164 DHRS-32-A---(0):1 ↔ DIN EN ISO 8734 4 x 10 - A:2
- Einfügen:7 [Insert]: 1310164 DHRS-32-A---(0):1 ↔ DIN EN ISO 8734 4 x 10 - A:1
- [Mate]: DIN 125 - A 5,3:1 ↔ DIN EN ISO 4762 - M5 x 10:1
- [Mate]: DIN 125 - A 5,3:1 ↔ DIN EN ISO 4762 - M5 x 10:1
- Passend:162 [Mate]: 1310164 DHRS-32-A---(0):1 ↔ DIN EN ISO 4762 - M5 x 10:1
- Passend:163 [Mate]: TS_Adapter_Greifer_int:1 ↔ DIN 125 - A 5,3:1
## Named parameters: Magazin_Hoehe = 255 mm, Abstand_Schrauben_vert = 105 mm, Abstand_Rand = 45 mm, Anbindung_Zylinder = 16.4 mm, d734_d646_d637_d627 = 0 mm, d735_d647_d641 = 0 mm
